# Autodesk Inventor assembly: assembly
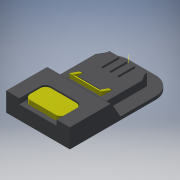
[picture p0: Inventor's stored thumbnail of the model, 180x180]
Saved by Autodesk Inventor 2016 (Build 200138000, 138)
## iProperties
Created: 2016-06-09
Part Number: assembly
Document SubType Name: Assembly
Designer: Chris
Author: Chris
## Documents named in this file (3)
- F:\projects\160609 gruetzkopf akku\assembly.iam
- F:\projects\160609 gruetzkopf akku\gehaeuse.ipt
- F:\projects\160609 gruetzkopf akku\schnapper.ipt
## Components (2 placed, 2 different names)
1. gehaeuse:1 — Flush:1, Flush:2, Flush:3
2. schnapper:1 — Flush:1, Flush:2, Flush:3
## Relationships (3: Flush 3)
- Flush:1: gehaeuse:1 ↔ schnapper:1
- Flush:2: gehaeuse:1 ↔ schnapper:1
- Flush:3 (0.5 mm): gehaeuse:1 ↔ schnapper:1
